# Autodesk Inventor assembly: ASM_Y-Axis
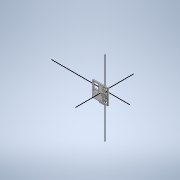
[picture p0: Inventor's stored thumbnail of the model, 180x180]
Saved by Autodesk Inventor 2022.2 (Build 262287010, 287A)
## iProperties
Created: 2024-09-30
Part Number: ASM_Y-Axis
Document SubType Name: Assembly
Designer: ppovolni
Author: ppovolni
## Documents named in this file (4)
- D:\3_Local_Projekte\_PaperGitHub\MiniBumblebee_LowFieldMapping\2_Calibration\21_Hardware\213_CalibrationSolenoid_CAD\Slider\Hallsensor_Mounting\Y-Axis\ASM_Y-Axis.iam
- D:\3_Local_Projekte\_PaperGitHub\MiniBumblebee_LowFieldMapping\2_Calibration\21_Hardware\213_CalibrationSolenoid_CAD\Slider\Hallsensor_Mounting\Y-Axis\HallSensor_Holder_Y-Axis.ipt
- D:\3_Local_Projekte\_PaperGitHub\MiniBumblebee_LowFieldMapping\2_Calibration\21_Hardware\213_CalibrationSolenoid_CAD\Slider\Hallsensor_Mounting\ASM_SensorHead_LowerSensor.iam
- D:\3_Local_Projekte\_PaperGitHub\MiniBumblebee_LowFieldMapping\2_Calibration\21_Hardware\213_CalibrationSolenoid_CAD\Slider\Hallsensor_Mounting\ASM_SensorHead_UpperSensor.iam
## Components (5 placed, 3 different names)
1. HallSensor_Holder_Y-Axis:1 — Winkel:1, Winkel:2, Passend:1, Passend:2, Passend:3, Passend:4, Passend:5
2. ASM_SensorHead_LowerSensor:2 [sub-assembly] — Fluchtend:1, Fluchtend:2, Passend:3, Fluchtend:3, Fluchtend:4
3. ASM_SensorHead_LowerSensor:1 [sub-assembly] — Winkel:1, Winkel:2, Passend:1, Passend:2, Fluchtend:1, Fluchtend:2
4. ASM_SensorHead_UpperSensor:1 [sub-assembly] — Fluchtend:3, Fluchtend:4, Passend:4, Fluchtend:5, Fluchtend:6
5. ASM_SensorHead_UpperSensor:2 [sub-assembly] — Fluchtend:5, Fluchtend:6, Passend:5
## Relationships (13: Flush 6, Mate 5, Angle 2)
- Winkel:1 [Angle] (0 deg): HallSensor_Holder_Y-Axis:1 ↔ ASM_SensorHead_LowerSensor:1
- Winkel:2 [Angle] (0 deg): HallSensor_Holder_Y-Axis:1 ↔ ASM_SensorHead_LowerSensor:1
- Passend:1 [Mate] (0.5 mm): HallSensor_Holder_Y-Axis:1 ↔ ASM_SensorHead_LowerSensor:1
- Passend:2 [Mate]: HallSensor_Holder_Y-Axis:1 ↔ ASM_SensorHead_LowerSensor:1
- Fluchtend:1 [Flush]: ASM_SensorHead_LowerSensor:2 ↔ ASM_SensorHead_LowerSensor:1
- Fluchtend:2 [Flush]: ASM_SensorHead_LowerSensor:2 ↔ ASM_SensorHead_LowerSensor:1
- Passend:3 [Mate]: HallSensor_Holder_Y-Axis:1 ↔ ASM_SensorHead_LowerSensor:2
- Fluchtend:3 [Flush]: ASM_SensorHead_LowerSensor:2 ↔ ASM_SensorHead_UpperSensor:1
- Fluchtend:4 [Flush]: ASM_SensorHead_LowerSensor:2 ↔ ASM_SensorHead_UpperSensor:1
- Passend:4 [Mate] (0.5 mm): HallSensor_Holder_Y-Axis:1 ↔ ASM_SensorHead_UpperSensor:1
- Fluchtend:5 [Flush]: ASM_SensorHead_UpperSensor:1 ↔ ASM_SensorHead_UpperSensor:2
- Fluchtend:6 [Flush]: ASM_SensorHead_UpperSensor:1 ↔ ASM_SensorHead_UpperSensor:2
- Passend:5 [Mate]: HallSensor_Holder_Y-Axis:1 ↔ ASM_SensorHead_UpperSensor:2
